# Autodesk Inventor assembly: TankFlipperAssembledDriveShaft
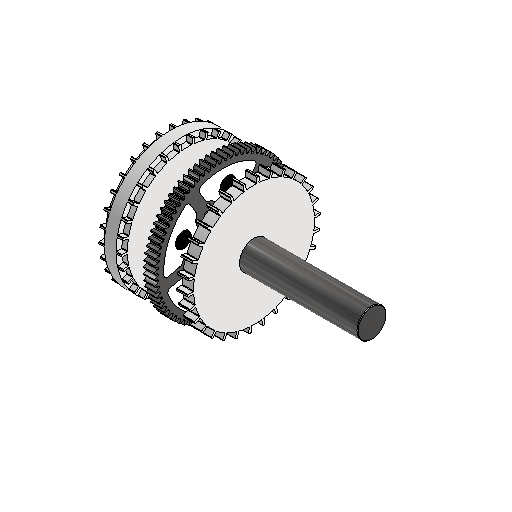
[picture p0: Inventor's stored thumbnail of the model, 512x512]
Saved by Autodesk Inventor 2025 (Build 290162000, 162)
## iProperties
Created: 2024-02-13
Part Number: TankFlipperAssembledDriveShaft
Document SubType Name: Assembly
Designer: seene
Author: seene
## Documents named in this file (14)
- C:\Users\seene\OneDrive\SBRT\Robocup Rescue\Drive\v1\TANK flipper\TankFlipperAssembledDriveShaft.iam
- C:\Users\seene\OneDrive\SBRT\Robocup Rescue\Drive\v1\TANK flipper\Drive Shaft.ipt
- C:\Users\seene\OneDrive\SBRT\Robocup Rescue\Drive\v1\TANK flipper\98585A121_Heavy Duty External Retaining Ring v2.ipt
- C:\Users\seene\OneDrive\SBRT\Robocup Rescue\Drive\v1\TANK flipper\2868T199_High-Load Oil-Embedded 863 Sleeve Bearing (1) v2(Mirror).ipt
- C:\Users\seene\OneDrive\SBRT\Robocup Rescue\Drive\v1\TANK flipper\Spur Gear (74 teeth).ipt
- C:\Users\seene\OneDrive\SBRT\Robocup Rescue\Drive\v1\TANK flipper\panel_flange.ipt
- C:\Users\seene\OneDrive\SBRT\Robocup Rescue\Drive\v1\TANK flipper\spacer_flange.ipt
- C:\Users\seene\OneDrive\SBRT\Robocup Rescue\Drive\v1\TANK flipper\transfer_pin.ipt
- C:\Users\seene\OneDrive\SBRT\Robocup Rescue\Drive\v1\TANK flipper\.25-20_FHCS_91263A553.ipt
- C:\Users\seene\OneDrive\SBRT\Robocup Rescue\Drive\v1\TANK flipper\bushing_2868T199.ipt
- C:\Users\seene\OneDrive\SBRT\Robocup Rescue\Drive\v1\TANK flipper\94328A911_Black Oxide Alloy Steel Low-Profile Shoulder Screw v2.ipt
- C:\Users\seene\OneDrive\SBRT\Robocup Rescue\Drive\v1\TANK flipper\FlipperSpurGearMount.ipt
- C:\Users\seene\OneDrive\SBRT\Robocup Rescue\Drive\v1\VTR-037_pulley.ipt
- C:\Users\seene\OneDrive\SBRT\Robocup Rescue\Drive\v1\TANK flipper\VTR-008_BigPulley.ipt
## Components (30 placed, 13 different names)
1. Drive Shaft:1 — Rigid:1, Rigid:2, Rigid:3, Rigid:5, Rigid:17, Mate:9, Mate:12, Mate:14
2. 98585A121_Heavy Duty External Retaining Ring v2:1 — Rigid:1
3. 2868T199_High-Load Oil-Embedded 863 Sleeve Bearing (1) v2(Mirror):1 — Rigid:2, Rigid:18
4. 98585A121_Heavy Duty External Retaining Ring v2:2 — Rigid:3
5. 98585A121_Heavy Duty External Retaining Ring v2:3 — Rigid:5
6. Spur Gear (74 teeth):1 — Mate:1, Mate:2, Mate:6, Mate:7, Mate:8, Mate:9, Mate:15
7. panel_flange:1 — Rigid:18, Mate:13
8. panel_flange:2 — Mate:3, Mate:4, Mate:5, Rigid:25, Mate:16
9. bushing_2868T199:1 — Rigid:26, Mate:1, Flush:2
10. bushing_2868T199:2 — Rigid:26
11. bushing_2868T199:3 — Rigid:17, Rigid:25
12. FlipperSpurGearMount:1 — Mate:6, Mate:7, Mate:8, Mate:10, Mate:11, Mate:16, Flush:2
13. VTR-037_pulley:1 — Mate:12, Mate:15
14. VTR-008_pulley:1 — Mate:13, Mate:14
15. transfer_pin:1 — Rigid:8
16. transfer_pin:2 — Rigid:9
17. transfer_pin:3 — Rigid:7
18. transfer_pin:4 — Rigid:10
19. transfer_pin:5 — Rigid:6
20. spacer_flange:1 — Rigid:6, Rigid:7, Rigid:8, Rigid:9, Rigid:10, Mate:2, Rigid:20, Rigid:21, Rigid:22, Rigid:23, Rigid:24
21. 94328A911_Black Oxide Alloy Steel Low-Profile Shoulder Screw v2:1 — Rigid:23, Mate:5
22. 94328A911_Black Oxide Alloy Steel Low-Profile Shoulder Screw v2:2 — Rigid:24
23. 94328A911_Black Oxide Alloy Steel Low-Profile Shoulder Screw v2:3 — Rigid:20
24. 94328A911_Black Oxide Alloy Steel Low-Profile Shoulder Screw v2:4 — Rigid:21, Mate:3, Mate:4
25. 94328A911_Black Oxide Alloy Steel Low-Profile Shoulder Screw v2:5 — Rigid:22
26. .25-20_FHCS_91263A553:1 — Mate:10, Mate:11
27. .25-20_FHCS_91263A553:2
28. .25-20_FHCS_91263A553:3
29. .25-20_FHCS_91263A553:4
30. .25-20_FHCS_91263A553:5
## Component patterns: (5 elements, first: .25-20_FHCS_91263A553:1)
## Relationships (35: WeldJoint 18, Mate 16, Flush 1)
- Rigid:1 [WeldJoint]: Drive Shaft:1 ↔ 98585A121_Heavy Duty External Retaining Ring v2:1
- Rigid:2 [WeldJoint]: Drive Shaft:1 ↔ 2868T199_High-Load Oil-Embedded 863 Sleeve Bearing (1) v2(Mirror):1
- Rigid:3 [WeldJoint]: Drive Shaft:1 ↔ 98585A121_Heavy Duty External Retaining Ring v2:2
- Rigid:5 [WeldJoint]: Drive Shaft:1 ↔ 98585A121_Heavy Duty External Retaining Ring v2:3
- Rigid:6 [WeldJoint]: transfer_pin:5 ↔ spacer_flange:1
- Rigid:7 [WeldJoint]: transfer_pin:3 ↔ spacer_flange:1
- Rigid:8 [WeldJoint]: transfer_pin:1 ↔ spacer_flange:1
- Rigid:9 [WeldJoint]: transfer_pin:2 ↔ spacer_flange:1
- Rigid:10 [WeldJoint]: transfer_pin:4 ↔ spacer_flange:1
- Mate:1: Spur Gear (74 teeth):1 ↔ bushing_2868T199:1
- Mate:2: Spur Gear (74 teeth):1 ↔ spacer_flange:1
- Rigid:17 [WeldJoint]: Drive Shaft:1 ↔ bushing_2868T199:3
- Rigid:18 [WeldJoint]: 2868T199_High-Load Oil-Embedded 863 Sleeve Bearing (1) v2(Mirror):1 ↔ panel_flange:1
- Rigid:20 [WeldJoint]: spacer_flange:1 ↔ 94328A911_Black Oxide Alloy Steel Low-Profile Shoulder Screw v2:3
- Rigid:21 [WeldJoint]: spacer_flange:1 ↔ 94328A911_Black Oxide Alloy Steel Low-Profile Shoulder Screw v2:4
- Rigid:22 [WeldJoint]: spacer_flange:1 ↔ 94328A911_Black Oxide Alloy Steel Low-Profile Shoulder Screw v2:5
- Rigid:23 [WeldJoint]: spacer_flange:1 ↔ 94328A911_Black Oxide Alloy Steel Low-Profile Shoulder Screw v2:1
- Rigid:24 [WeldJoint]: spacer_flange:1 ↔ 94328A911_Black Oxide Alloy Steel Low-Profile Shoulder Screw v2:2
- Mate:3: panel_flange:2 ↔ 94328A911_Black Oxide Alloy Steel Low-Profile Shoulder Screw v2:4
- Mate:4: panel_flange:2 ↔ 94328A911_Black Oxide Alloy Steel Low-Profile Shoulder Screw v2:4
- Mate:5: panel_flange:2 ↔ 94328A911_Black Oxide Alloy Steel Low-Profile Shoulder Screw v2:1
- Rigid:25 [WeldJoint]: panel_flange:2 ↔ bushing_2868T199:3
- Rigid:26 [WeldJoint]: bushing_2868T199:1 ↔ bushing_2868T199:2
- Mate:6: Spur Gear (74 teeth):1 ↔ FlipperSpurGearMount:1
- Mate:7: Spur Gear (74 teeth):1 ↔ FlipperSpurGearMount:1
- Mate:8: Spur Gear (74 teeth):1 ↔ FlipperSpurGearMount:1
- Mate:9: Drive Shaft:1 ↔ Spur Gear (74 teeth):1
- Mate:10: FlipperSpurGearMount:1 ↔ .25-20_FHCS_91263A553:1
- Mate:11: FlipperSpurGearMount:1 ↔ .25-20_FHCS_91263A553:1
- Mate:16 (6.35 mm): panel_flange:2 ↔ FlipperSpurGearMount:1
- Mate:12: Drive Shaft:1 ↔ VTR-037_pulley:1
- Mate:13 (5.4432 mm): panel_flange:1 ↔ VTR-008_pulley:1
- Mate:14: Drive Shaft:1 ↔ VTR-008_pulley:1
- Mate:15 (17.145 mm): Spur Gear (74 teeth):1 ↔ VTR-037_pulley:1
- Flush:2: bushing_2868T199:1 ↔ FlipperSpurGearMount:1
